# Autodesk Inventor assembly: A_Drive
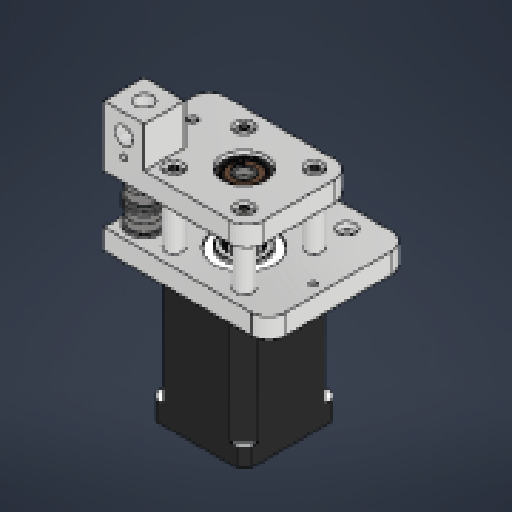
[picture p0: Inventor's stored thumbnail of the model, 512x512]
Saved by Autodesk Inventor 2026 (Build 300175050, 175E)
## iProperties
Created: 2025-05-23
Part Number: A_Drive
Document SubType Name: Assembly
Designer: Joshua Eah
Author: Joshua Eah
## Documents named in this file (14)
- C:\Users\Joshua Eah\Documents\GitHub\Voron-0\CAD\Tulip - Machined Parts\AB Drives\A Drive\A_Drive.iam
- C:\Users\Joshua Eah\Documents\GitHub\Voron-0\CAD\Tulip - Machined Parts\AB Drives\A Drive\A Drive Frame Upper (Tulip).ipt
- C:\Users\Joshua Eah\Documents\GitHub\Voron-0\CAD\Tulip - Machined Parts\AB Drives\A Drive\A Drive Frame Lower (Tulip).ipt
- C:\Users\Joshua Eah\Documents\GitHub\Voron-0\CAD\Master Assembly\Hardware\M3x10 BHCS.ipt
- C:\Users\Joshua Eah\Documents\GitHub\Voron-0\CAD\Master Assembly\Hardware\M3x30 BHCS.ipt
- C:\Users\Joshua Eah\Documents\GitHub\Voron-0\CAD\Master Assembly\Hardware\M3_Washer.ipt
- C:\Users\Joshua Eah\Documents\GitHub\Voron-0\CAD\Master Assembly\Hardware\3x30 Pin.ipt
- C:\Users\Joshua Eah\Documents\GitHub\Voron-0\CAD\Master Assembly\Hardware\F623 Stack.iam
- C:\Users\Joshua Eah\Documents\GitHub\Voron-0\CAD\Machined Parts\Spacers\Spacer.ipt
- C:\Users\Joshua Eah\Documents\GitHub\Voron-0\CAD\Tulip - Machined Parts\AB Drives\Drive Frame Spacer\Drive Frame Spacer.ipt
- C:\Users\Joshua Eah\Documents\GitHub\Voron-0\CAD\Master Assembly\AB Drives\Motor Assembly\Nema14.ipt
- C:\Users\Joshua Eah\Documents\GitHub\Voron-0\CAD\Master Assembly\Hardware\GT2 20T 6mm Pulley.iam
- C:\Users\Joshua Eah\Documents\GitHub\Voron-0\CAD\Master Assembly\Hardware\625ZZ Bearing.iam
- 625ZZ Bearing.iam
## Components (25 placed, 12 different names)
1. A Drive Frame Upper (Tulip):1 — Insert:2, Insert:8, Insert:9, Insert:10, Insert:11, Mate:2, Mate:3, Insert:16, Insert:24
2. A Drive Frame Lower (Tulip):1 — Insert:3, Insert:14, Insert:15, Insert:12, Mate:6, Insert:18, Insert:19, Insert:20, Insert:21
3. GT2 20T 6mm Pulley:1 [sub-assembly]
4. 625ZZ Bearing:1 [sub-assembly] — Insert:24
5. Nema14:1
6. M3x10 BHCS:1 — Insert:2
7. M3x10 BHCS:2 — Insert:3
8. M3x30 BHCS:1 — Insert:4
9. M3_Washer:1 — Insert:4, Insert:8
10. M3x30 BHCS:2
11. M3_Washer:2 — Insert:9
12. M3x30 BHCS:3
13. M3_Washer:3 — Insert:10
14. M3x30 BHCS:4
15. M3_Washer:4 — Insert:11
16. 3x30 Pin:1 — Mate:2, Insert:14
17. 3x30 Pin:2 — Mate:3, Insert:15
18. F623 Stack:1 [sub-assembly] — Insert:12, Insert:17
19. F623 Stack:2 [sub-assembly] — Mate:6, Insert:13
20. F623 Stack:3 [sub-assembly] — Insert:13, Insert:16
21. Spacer:1 — Insert:17
22. Drive Frame Spacer:1 — Insert:18
23. Drive Frame Spacer:2 — Insert:19
24. Drive Frame Spacer:3 — Insert:20
25. Drive Frame Spacer:4 — Insert:21
## Relationships (24: Insert 21, Mate 3)
- Insert:2: A Drive Frame Upper (Tulip):1 ↔ M3x10 BHCS:1
- Insert:3: A Drive Frame Lower (Tulip):1 ↔ M3x10 BHCS:2
- Insert:4: M3x30 BHCS:1 ↔ M3_Washer:1
- [Insert]: M3x30 BHCS:2 ↔ M3_Washer:2
- [Insert]: M3x30 BHCS:3 ↔ M3_Washer:3
- [Insert]: M3x30 BHCS:4 ↔ M3_Washer:4
- Insert:8: A Drive Frame Upper (Tulip):1 ↔ M3_Washer:1
- Insert:9: A Drive Frame Upper (Tulip):1 ↔ M3_Washer:2
- Insert:10: A Drive Frame Upper (Tulip):1 ↔ M3_Washer:3
- Insert:11: A Drive Frame Upper (Tulip):1 ↔ M3_Washer:4
- Mate:2: A Drive Frame Upper (Tulip):1 ↔ 3x30 Pin:1
- Mate:3: A Drive Frame Upper (Tulip):1 ↔ 3x30 Pin:2
- Insert:14: A Drive Frame Lower (Tulip):1 ↔ 3x30 Pin:1
- Insert:15: A Drive Frame Lower (Tulip):1 ↔ 3x30 Pin:2
- Insert:12: A Drive Frame Lower (Tulip):1 ↔ F623 Stack:1
- Mate:6: A Drive Frame Lower (Tulip):1 ↔ F623 Stack:2
- Insert:13: F623 Stack:2 ↔ F623 Stack:3
- Insert:16: A Drive Frame Upper (Tulip):1 ↔ F623 Stack:3
- Insert:17: F623 Stack:1 ↔ Spacer:1
- Insert:18: A Drive Frame Lower (Tulip):1 ↔ Drive Frame Spacer:1
- Insert:19: A Drive Frame Lower (Tulip):1 ↔ Drive Frame Spacer:2
- Insert:20: A Drive Frame Lower (Tulip):1 ↔ Drive Frame Spacer:3
- Insert:21: A Drive Frame Lower (Tulip):1 ↔ Drive Frame Spacer:4
- Insert:24: A Drive Frame Upper (Tulip):1 ↔ 625ZZ Bearing:1
## Named parameters: d9_d8 = 0 mm, d10_d8 = 0 mm, d11_d8 = 0 mm
